# Autodesk Inventor assembly: 000-ball_loading_v1
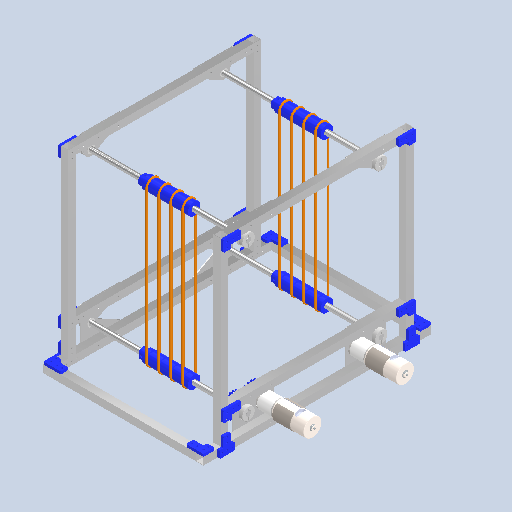
[picture p0: Inventor's stored thumbnail of the model, 512x512]
Saved by Autodesk Inventor 2025.1 (Build 291241000, 241)
## iProperties
Created: 2024-11-12
Part Number: 000-ball_loading_v1
Document SubType Name: Assembly
Designer: haruy
Author: haruy
## Documents named in this file (19)
- C:\Users\haruy\Documents\ロボコン\NHK2025\cad\nagahisa\ball_loading\000-ball_loading_v1.iam
- C:\Users\haruy\Documents\ロボコン\NHK2025\cad\nagahisa\ball_loading\ball_loading_v1_ASP_Base.ipt
- C:\Users\haruy\Documents\ロボコン\NHK2025\cad\nagahisa\ball_loading\ball_loading_v1_Plate_up_F.ipt
- C:\Users\haruy\Documents\ロボコン\NHK2025\cad\nagahisa\ball_loading\ball_loading_v1_Plate_right_down_M_F.ipt
- C:\Users\haruy\Documents\ロボコン\NHK2025\cad\000_parts\モーター\mabuchi 555+IG32.iam
- C:\Users\haruy\Documents\ロボコン\NHK2025\cad\000_parts\ベアリング\10\bear_10_15_sn.ipt
- C:\Users\haruy\Documents\ロボコン\NHK2025\cad\nagahisa\ball_loading\ball_loading_v1_Plate_right_down_R_F.ipt
- C:\Users\haruy\Documents\ロボコン\NHK2025\cad\nagahisa\ball_loading\ball_loading_v1_Plate_left_up_F.ipt
- C:\Users\haruy\Documents\ロボコン\NHK2025\cad\nagahisa\ball_loading\ball_loading_v1_Plate_left_down_M_F.ipt
- C:\Users\haruy\Documents\ロボコン\NHK2025\cad\nagahisa\ball_loading\ball_loading_v1_Plate_left_down_R_F.ipt
- C:\Users\haruy\Documents\ロボコン\NHK2025\cad\nagahisa\ball_loading\ball_loading_v1_Plate_ASP_F_1.ipt
- C:\Users\haruy\Documents\ロボコン\NHK2025\cad\nagahisa\ball_loading\ball_loading_v1_Plate_ASP_F_2.ipt
- C:\Users\haruy\Documents\ロボコン\NHK2025\cad\nagahisa\ball_loading\ball_loading_v1_Plate_ASP_F_3.ipt
- C:\Users\haruy\Documents\ロボコン\NHK2025\cad\nagahisa\ball_loading\ball_loading_v1_Shaft_1.ipt
- C:\Users\haruy\Documents\ロボコン\NHK2025\cad\nagahisa\ball_loading\PSCBNJ10-13b.ipt
- C:\Users\haruy\Documents\ロボコン\NHK2025\cad\nagahisa\ball_loading\ball_loading_v1_3DP_P_B.ipt
- C:\Users\haruy\Documents\ロボコン\NHK2025\cad\nagahisa\ball_loading\ball_loading_v1_circle_B.ipt
- C:\Users\haruy\Documents\ロボコン\NHK2025\cad\nagahisa\hand\roller\SCSWJ6-6_b.ipt
- C:\Users\haruy\Documents\ロボコン\NHK2025\cad\nagahisa\ball_loading\000-ball_loading_v1\デザイン アクセラレータ\平歯車1.iam
## Components (56 placed, 18 different names)
1. ball_loading_v1_ASP_Base:1 — 挿入:1, 挿入:2, 挿入:3, 挿入:4, 挿入:5, 挿入:6, 挿入:11, 挿入:12, 挿入:14, 挿入:15, 挿入:16, 挿入:17, 挿入:20, 挿入:21, 挿入:22, 挿入:23, 挿入:27, 挿入:28, 挿入:29, 挿入:30, 挿入:31, 挿入:32, 挿入:33, 挿入:34, 挿入:35, 挿入:36, 挿入:37, 挿入:38, 挿入:39, 挿入:40, 挿入:41, 挿入:42, 挿入:43, 挿入:44, 挿入:45, 挿入:46, 挿入:47, 挿入:48, 挿入:49, 挿入:50, 挿入:51, 挿入:52, 挿入:53, 挿入:54, 挿入:55, 挿入:56, 挿入:57, 挿入:58
2. ball_loading_v1_Plate_up_F:1 — 挿入:1, 挿入:2, 挿入:9
3. ball_loading_v1_Plate_up_F:2 — 挿入:3, 挿入:4, 挿入:10
4. ball_loading_v1_Plate_right_down_M_F:1 — 挿入:5, 挿入:6, 挿入:7, 挿入:8
5. mabuchi 555+IG32:1 [sub-assembly] — 挿入:7, 挿入:79, メイト:1
6. bear_10_15_sn:1 — 挿入:8, 挿入:63
7. bear_10_15_sn:2 — 挿入:9, 挿入:64
8. bear_10_15_sn:3 — 挿入:10, 挿入:60, 挿入:68, 挿入:72
9. ball_loading_v1_Plate_right_down_R_F:1 — 挿入:11, 挿入:12, 挿入:13
10. bear_10_15_sn:4 — 挿入:13, 挿入:59, 挿入:67, 挿入:71
11. ball_loading_v1_Plate_left_up_F:1 — 挿入:14, 挿入:15, 挿入:18
12. ball_loading_v1_Plate_left_up_F:2 — 挿入:16, 挿入:17, 挿入:19
13. bear_10_15_sn:5 — 挿入:18, 挿入:66
14. bear_10_15_sn:6 — 挿入:19, 挿入:61, 挿入:70, 挿入:74
15. ball_loading_v1_Plate_left_down_M_F:1 — 挿入:20, 挿入:21, 挿入:24, 挿入:26
16. ball_loading_v1_Plate_left_down_R_F:1 — 挿入:22, 挿入:23, 挿入:25
17. bear_10_15_sn:7 — 挿入:24, 挿入:65
18. bear_10_15_sn:8 — 挿入:25, 挿入:62, 挿入:69, 挿入:73
19. mabuchi 555+IG32:2 [sub-assembly] — 挿入:26, 挿入:80
20. ball_loading_v1_Plate_ASP_F_1:1 — 挿入:27, 挿入:28
21. ball_loading_v1_Plate_ASP_F_1:2 — 挿入:29, 挿入:30
22. ball_loading_v1_Plate_ASP_F_1:3 — 挿入:31, 挿入:32
23. ball_loading_v1_Plate_ASP_F_1:4 — 挿入:33, 挿入:34
24. ball_loading_v1_Plate_ASP_F_2:1 — 挿入:35, 挿入:36
25. ball_loading_v1_Plate_ASP_F_2:2 — 挿入:37, 挿入:38
26. ball_loading_v1_Plate_ASP_F_2:3 — 挿入:41, 挿入:42
27. ball_loading_v1_Plate_ASP_F_2:4 — 挿入:39, 挿入:40
28. ball_loading_v1_Plate_ASP_F_2:5 — 挿入:43, 挿入:44
29. ball_loading_v1_Plate_ASP_F_2:6 — 挿入:45, 挿入:46
30. ball_loading_v1_Plate_ASP_F_2:7 — 挿入:47, 挿入:48
31. ball_loading_v1_Plate_ASP_F_2:8 — 挿入:49, 挿入:50
32. ball_loading_v1_Plate_ASP_F_3:1 — 挿入:51, 挿入:52
33. ball_loading_v1_Plate_ASP_F_3:2 — 挿入:53, 挿入:54
34. ball_loading_v1_Plate_ASP_F_3:3 — 挿入:55, 挿入:56
35. ball_loading_v1_Plate_ASP_F_3:4 — 挿入:57, 挿入:58
36. ball_loading_v1_Shaft_1:1 — 挿入:59, メイト:3
37. ball_loading_v1_Shaft_1:2 — 挿入:60
38. ball_loading_v1_Shaft_1:3 — 挿入:61
39. ball_loading_v1_Shaft_1:4 — 挿入:62
40. PSCBNJ10-13b:1 — 挿入:63
41. PSCBNJ10-13b:2 — 挿入:66
42. PSCBNJ10-13b:3 — 挿入:65
43. PSCBNJ10-13b:4 — 挿入:64
44. PSCBNJ10-13b:5 — 挿入:67
45. PSCBNJ10-13b:6 — 挿入:68
46. PSCBNJ10-13b:7 — 挿入:69
47. PSCBNJ10-13b:8 — 挿入:70
48. ball_loading_v1_3DP_P_B:1 — 挿入:73, 挿入:77
49. ball_loading_v1_3DP_P_B:2 — 挿入:74, 挿入:78
50. ball_loading_v1_3DP_P_B:3 — 挿入:72, 挿入:76
51. ball_loading_v1_3DP_P_B:4 — 挿入:71, 挿入:75
52. ball_loading_v1_circle_B:1 — 挿入:75, 挿入:76
53. ball_loading_v1_circle_B:2 — 挿入:77, 挿入:78
54. SCSWJ6-6_b:1 — 挿入:79, メイト:2
55. SCSWJ6-6_b:2 — 挿入:80
56. 平歯車:1 [sub-assembly] — メイト:1, メイト:2, メイト:3
## Relationships (83: Insert 80, Mate 3)
- 挿入:1 [Insert]: ball_loading_v1_ASP_Base:1 ↔ ball_loading_v1_Plate_up_F:1
- 挿入:2 [Insert]: ball_loading_v1_ASP_Base:1 ↔ ball_loading_v1_Plate_up_F:1
- 挿入:3 [Insert]: ball_loading_v1_ASP_Base:1 ↔ ball_loading_v1_Plate_up_F:2
- 挿入:4 [Insert]: ball_loading_v1_ASP_Base:1 ↔ ball_loading_v1_Plate_up_F:2
- 挿入:5 [Insert]: ball_loading_v1_ASP_Base:1 ↔ ball_loading_v1_Plate_right_down_M_F:1
- 挿入:6 [Insert]: ball_loading_v1_ASP_Base:1 ↔ ball_loading_v1_Plate_right_down_M_F:1
- 挿入:7 [Insert]: ball_loading_v1_Plate_right_down_M_F:1 ↔ mabuchi 555+IG32:1
- 挿入:8 [Insert]: ball_loading_v1_Plate_right_down_M_F:1 ↔ bear_10_15_sn:1
- 挿入:9 [Insert]: ball_loading_v1_Plate_up_F:1 ↔ bear_10_15_sn:2
- 挿入:10 [Insert]: ball_loading_v1_Plate_up_F:2 ↔ bear_10_15_sn:3
- 挿入:11 [Insert]: ball_loading_v1_ASP_Base:1 ↔ ball_loading_v1_Plate_right_down_R_F:1
- 挿入:12 [Insert]: ball_loading_v1_ASP_Base:1 ↔ ball_loading_v1_Plate_right_down_R_F:1
- 挿入:13 [Insert]: ball_loading_v1_Plate_right_down_R_F:1 ↔ bear_10_15_sn:4
- 挿入:14 [Insert]: ball_loading_v1_ASP_Base:1 ↔ ball_loading_v1_Plate_left_up_F:1
- 挿入:15 [Insert]: ball_loading_v1_ASP_Base:1 ↔ ball_loading_v1_Plate_left_up_F:1
- 挿入:16 [Insert]: ball_loading_v1_ASP_Base:1 ↔ ball_loading_v1_Plate_left_up_F:2
- 挿入:17 [Insert]: ball_loading_v1_ASP_Base:1 ↔ ball_loading_v1_Plate_left_up_F:2
- 挿入:18 [Insert]: ball_loading_v1_Plate_left_up_F:1 ↔ bear_10_15_sn:5
- 挿入:19 [Insert]: ball_loading_v1_Plate_left_up_F:2 ↔ bear_10_15_sn:6
- 挿入:20 [Insert]: ball_loading_v1_ASP_Base:1 ↔ ball_loading_v1_Plate_left_down_M_F:1
- 挿入:21 [Insert]: ball_loading_v1_ASP_Base:1 ↔ ball_loading_v1_Plate_left_down_M_F:1
- 挿入:22 [Insert]: ball_loading_v1_ASP_Base:1 ↔ ball_loading_v1_Plate_left_down_R_F:1
- 挿入:23 [Insert]: ball_loading_v1_ASP_Base:1 ↔ ball_loading_v1_Plate_left_down_R_F:1
- 挿入:24 [Insert]: ball_loading_v1_Plate_left_down_M_F:1 ↔ bear_10_15_sn:7
- 挿入:25 [Insert]: ball_loading_v1_Plate_left_down_R_F:1 ↔ bear_10_15_sn:8
- 挿入:26 [Insert]: ball_loading_v1_Plate_left_down_M_F:1 ↔ mabuchi 555+IG32:2
- 挿入:27 [Insert]: ball_loading_v1_ASP_Base:1 ↔ ball_loading_v1_Plate_ASP_F_1:1
- 挿入:28 [Insert]: ball_loading_v1_ASP_Base:1 ↔ ball_loading_v1_Plate_ASP_F_1:1
- 挿入:29 [Insert]: ball_loading_v1_ASP_Base:1 ↔ ball_loading_v1_Plate_ASP_F_1:2
- 挿入:30 [Insert]: ball_loading_v1_ASP_Base:1 ↔ ball_loading_v1_Plate_ASP_F_1:2
- 挿入:31 [Insert]: ball_loading_v1_ASP_Base:1 ↔ ball_loading_v1_Plate_ASP_F_1:3
- 挿入:32 [Insert]: ball_loading_v1_ASP_Base:1 ↔ ball_loading_v1_Plate_ASP_F_1:3
- 挿入:33 [Insert]: ball_loading_v1_ASP_Base:1 ↔ ball_loading_v1_Plate_ASP_F_1:4
- 挿入:34 [Insert]: ball_loading_v1_ASP_Base:1 ↔ ball_loading_v1_Plate_ASP_F_1:4
- 挿入:35 [Insert]: ball_loading_v1_ASP_Base:1 ↔ ball_loading_v1_Plate_ASP_F_2:1
- 挿入:36 [Insert]: ball_loading_v1_ASP_Base:1 ↔ ball_loading_v1_Plate_ASP_F_2:1
- 挿入:37 [Insert]: ball_loading_v1_ASP_Base:1 ↔ ball_loading_v1_Plate_ASP_F_2:2
- 挿入:38 [Insert]: ball_loading_v1_ASP_Base:1 ↔ ball_loading_v1_Plate_ASP_F_2:2
- 挿入:39 [Insert]: ball_loading_v1_ASP_Base:1 ↔ ball_loading_v1_Plate_ASP_F_2:4
- 挿入:40 [Insert]: ball_loading_v1_ASP_Base:1 ↔ ball_loading_v1_Plate_ASP_F_2:4
- 挿入:41 [Insert]: ball_loading_v1_ASP_Base:1 ↔ ball_loading_v1_Plate_ASP_F_2:3
- 挿入:42 [Insert]: ball_loading_v1_ASP_Base:1 ↔ ball_loading_v1_Plate_ASP_F_2:3
- 挿入:43 [Insert]: ball_loading_v1_ASP_Base:1 ↔ ball_loading_v1_Plate_ASP_F_2:5
- 挿入:44 [Insert]: ball_loading_v1_ASP_Base:1 ↔ ball_loading_v1_Plate_ASP_F_2:5
- 挿入:45 [Insert]: ball_loading_v1_ASP_Base:1 ↔ ball_loading_v1_Plate_ASP_F_2:6
- 挿入:46 [Insert]: ball_loading_v1_ASP_Base:1 ↔ ball_loading_v1_Plate_ASP_F_2:6
- 挿入:47 [Insert]: ball_loading_v1_ASP_Base:1 ↔ ball_loading_v1_Plate_ASP_F_2:7
- 挿入:48 [Insert]: ball_loading_v1_ASP_Base:1 ↔ ball_loading_v1_Plate_ASP_F_2:7
- 挿入:49 [Insert]: ball_loading_v1_ASP_Base:1 ↔ ball_loading_v1_Plate_ASP_F_2:8
- 挿入:50 [Insert]: ball_loading_v1_ASP_Base:1 ↔ ball_loading_v1_Plate_ASP_F_2:8
- 挿入:51 [Insert]: ball_loading_v1_ASP_Base:1 ↔ ball_loading_v1_Plate_ASP_F_3:1
- 挿入:52 [Insert]: ball_loading_v1_ASP_Base:1 ↔ ball_loading_v1_Plate_ASP_F_3:1
- 挿入:53 [Insert]: ball_loading_v1_ASP_Base:1 ↔ ball_loading_v1_Plate_ASP_F_3:2
- 挿入:54 [Insert]: ball_loading_v1_ASP_Base:1 ↔ ball_loading_v1_Plate_ASP_F_3:2
- 挿入:55 [Insert]: ball_loading_v1_ASP_Base:1 ↔ ball_loading_v1_Plate_ASP_F_3:3
- 挿入:56 [Insert]: ball_loading_v1_ASP_Base:1 ↔ ball_loading_v1_Plate_ASP_F_3:3
- 挿入:57 [Insert]: ball_loading_v1_ASP_Base:1 ↔ ball_loading_v1_Plate_ASP_F_3:4
- 挿入:58 [Insert]: ball_loading_v1_ASP_Base:1 ↔ ball_loading_v1_Plate_ASP_F_3:4
- 挿入:59 [Insert] (-10 mm): bear_10_15_sn:4 ↔ ball_loading_v1_Shaft_1:1
- 挿入:60 [Insert] (-10 mm): bear_10_15_sn:3 ↔ ball_loading_v1_Shaft_1:2
- 挿入:61 [Insert] (-10 mm): bear_10_15_sn:6 ↔ ball_loading_v1_Shaft_1:3
- 挿入:62 [Insert] (-10 mm): bear_10_15_sn:8 ↔ ball_loading_v1_Shaft_1:4
- 挿入:63 [Insert]: bear_10_15_sn:1 ↔ PSCBNJ10-13b:1
- 挿入:64 [Insert]: bear_10_15_sn:2 ↔ PSCBNJ10-13b:4
- 挿入:65 [Insert]: bear_10_15_sn:7 ↔ PSCBNJ10-13b:3
- 挿入:66 [Insert]: bear_10_15_sn:5 ↔ PSCBNJ10-13b:2
- 挿入:67 [Insert]: bear_10_15_sn:4 ↔ PSCBNJ10-13b:5
- 挿入:68 [Insert]: bear_10_15_sn:3 ↔ PSCBNJ10-13b:6
- 挿入:69 [Insert]: bear_10_15_sn:8 ↔ PSCBNJ10-13b:7
- 挿入:70 [Insert]: bear_10_15_sn:6 ↔ PSCBNJ10-13b:8
- 挿入:71 [Insert] (103 mm): bear_10_15_sn:4 ↔ ball_loading_v1_3DP_P_B:4
- 挿入:72 [Insert] (103 mm): bear_10_15_sn:3 ↔ ball_loading_v1_3DP_P_B:3
- 挿入:73 [Insert] (103 mm): bear_10_15_sn:8 ↔ ball_loading_v1_3DP_P_B:1
- 挿入:74 [Insert] (103 mm): bear_10_15_sn:6 ↔ ball_loading_v1_3DP_P_B:2
- 挿入:75 [Insert] (20 mm): ball_loading_v1_3DP_P_B:4 ↔ ball_loading_v1_circle_B:1
- 挿入:76 [Insert] (20 mm): ball_loading_v1_3DP_P_B:3 ↔ ball_loading_v1_circle_B:1
- 挿入:77 [Insert] (20 mm): ball_loading_v1_3DP_P_B:1 ↔ ball_loading_v1_circle_B:2
- 挿入:78 [Insert] (20 mm): ball_loading_v1_3DP_P_B:2 ↔ ball_loading_v1_circle_B:2
- 挿入:79 [Insert] (5 mm): mabuchi 555+IG32:1 ↔ SCSWJ6-6_b:1
- 挿入:80 [Insert] (5 mm): mabuchi 555+IG32:2 ↔ SCSWJ6-6_b:2
- メイト:1 [Mate]: mabuchi 555+IG32:1 ↔ 平歯車:1
- メイト:2 [Mate]: SCSWJ6-6_b:1 ↔ 平歯車:1
- メイト:3 [Mate]: ball_loading_v1_Shaft_1:1 ↔ 平歯車:1
